# Autodesk Inventor assembly: Filament Runout Sensor Foot (1)
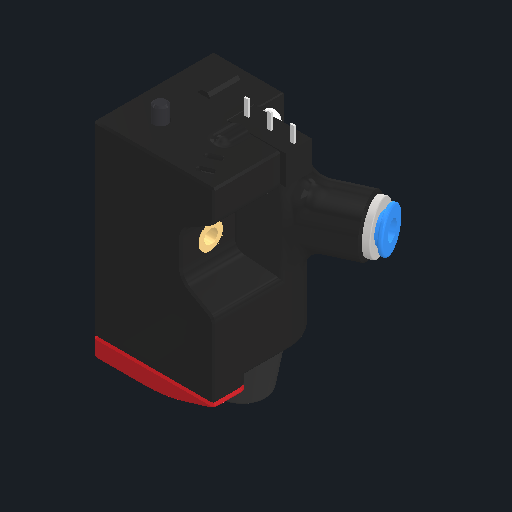
[picture p0: Inventor's stored thumbnail of the model, 512x512]
Saved by Autodesk Inventor 2025.1 (Build 291241020, 241B)
## iProperties
Created: 2025-05-09
Part Number: Filament Runout Sensor Foot (1)
Document SubType Name: Assembly
Designer: AdminForWorker
Title: Filament Runout Sensor Foot (1)
Author: AdminForWorker
## Documents named in this file (8)
- C:\Users\Joshua Eah\Documents\Voron 0.2\CAD\Master Assembly\Filament Runout Sensor Foot (1).iam
- C:\Users\Joshua Eah\Documents\Voron 0.2\CAD\Master Assembly\Printed Parts (28).iam
- C:\Users\Joshua Eah\Documents\Voron 0.2\CAD\Master Assembly\Hardware\Threaded Insert Assemblies\Threaded Inserts (3).iam
- C:\Users\Joshua Eah\Documents\Voron 0.2\CAD\Master Assembly\Runout Sensor Hardware.iam
- C:\Users\Joshua Eah\Documents\Voron 0.2\CAD\Master Assembly\Rubber Foot.ipt
- C:\Users\Joshua Eah\Documents\Voron 0.2\CAD\Master Assembly\Hardware\M2x10 Self Tapper.ipt
- C:\Users\Joshua Eah\Documents\Voron 0.2\CAD\Master Assembly\Hardware\M3x40 BHCS.ipt
- C:\Users\Joshua Eah\Documents\Voron 0.2\CAD\Master Assembly\Hardware\M3x10 BHCS.ipt
## Components (8 placed, 7 different names)
1. Printed Parts (28):1 [sub-assembly] — Insert:1, Insert:2
2. Threaded Inserts (3):1 [sub-assembly]
3. Runout Sensor Hardware:1 [sub-assembly]
4. Rubber Foot:4
5. M2x10 Self Tapper:1 — Insert:1
6. M2x10 Self Tapper:2 — Insert:2
7. M3x40 BHCS:1
8. M3x10 BHCS:1
## Relationships (2: Insert 2)
- Insert:1: Printed Parts (28):1 ↔ M2x10 Self Tapper:1
- Insert:2: Printed Parts (28):1 ↔ M2x10 Self Tapper:2
